# Autodesk Inventor assembly: assembled-antenna
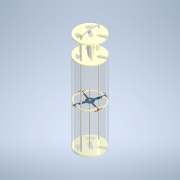
[picture p0: Inventor's stored thumbnail of the model, 180x180]
Saved by Autodesk Inventor 2021 (Build 250183000, 183)
## iProperties
Created: 2020-09-03
Part Number: assembled-antenna
Document SubType Name: Assembly
Designer: dsouthall
Author: dsouthall
## iProperties of the stored document inice_bottom.ipt
Created: 2020-11-16
Part Number: inice_bottom
Material: Generic
Document SubType Name: Modeling
Designer: dsouthall
Density: 1 g/cm^3
Appearance: Default
Author: dsouthall
Revision Number: ANY
## iProperties of the stored document inice_top.ipt
Created: 2020-11-16
Part Number: inice_top
Material: Generic
Document SubType Name: Modeling
Designer: dsouthall
Density: 1 g/cm^3
Appearance: Default
Author: dsouthall
Revision Number: ANY
## iProperties of the stored document front_end_box.iam
Created: 2020-11-16
Part Number: front_end_box
Description: STEP AP203
Document SubType Name: Assembly
Designer: dsouthall
Sending System: SolidWorks 2014
Preprocessor: SwSTEP 2.0
Title: front_end_box.STEP
Revision Number: ANY
## iProperties of the stored document fake_sma_with_cable.ipt
Created: 2020-11-16
Part Number: fake_sma_with_cable
Material: Generic
Document SubType Name: Modeling
Designer: dsouthall
Density: 1 g/cm^3
Appearance: Default
Author: dsouthall
Revision Number: ANY
## Documents named in this file (16)
- C:\Users\dsouthall\OneDrive - The University of Chicago\Hpol\hpol-prototype\design\Quad-Slot\Model 8 in\assembled-closed-antenna.iam
- C:\Users\dsouthall\OneDrive - The University of Chicago\Hpol\hpol-prototype\design\Quad-Slot\Model 8 in\assembled-feed.iam
- C:\Users\dsouthall\OneDrive - The University of Chicago\Hpol\hpol-prototype\design\Quad-Slot\Model 8 in\source\92141A003_TYPE 18-8 STAINLESS STEEL FLAT WASHER\92141A003_TYPE 18-8 STAINLESS STEEL FLAT WASHER.ipt
- C:\Users\dsouthall\OneDrive - The University of Chicago\Hpol\hpol-prototype\design\Quad-Slot\Model 8 in\source\96877A118_18-8 SS 82 DEG FLAT HEAD PHIL MACHINE SCREW\96877A118_18-8 SS 82 DEG FLAT HEAD PHIL MACHINE SCREW.ipt
- C:\Users\dsouthall\OneDrive - The University of Chicago\Hpol\hpol-prototype\design\Quad-Slot\Model 8 in\source\91841A003_TYPE 18-8 STAINLESS STEEL HEX NUT\91841A003_TYPE 18-8 STAINLESS STEEL HEX NUT.ipt
- C:\Users\dsouthall\OneDrive - The University of Chicago\Hpol\hpol-prototype\design\Quad-Slot\Model 8 in\source\my_faceplate.ipt
- C:\Users\dsouthall\OneDrive - The University of Chicago\Hpol\hpol-prototype\design\Quad-Slot\Model 8 in\source\my can\can_closed.ipt
- C:\Users\dsouthall\OneDrive - The University of Chicago\Hpol\hpol-prototype\design\Quad-Slot\Model 8 in\source\End Cap.ipt
- C:\Users\dsouthall\OneDrive - The University of Chicago\Hpol\hpol-prototype\design\Quad-Slot\Model 8 in\source\Short Support.ipt
- **C:\Users\dsouthall\OneDrive - The University of Chicago\Hpol\hpol-prototype\design\Quad-Slot\Model 8 in\assembled-closed-antenna.iam*LocalDocs*xAaaaamdaAaaaaaaaAaaaaxhxFa*front_end_box.iam
- C:\Users\dsouthall\OneDrive - The University of Chicago\Hpol\hpol-prototype\design\Quad-Slot\Model 8 in\source\rope.ipt
- C:\Users\dsouthall\OneDrive - The University of Chicago\Hpol\hpol-prototype\design\Quad-Slot\Model 8 in\source\99362A200_TAPPING INSERTS FOR PLASTICS\99362A200_TAPPING INSERTS FOR PLASTICS.ipt
- **C:\Users\dsouthall\OneDrive - The University of Chicago\Hpol\hpol-prototype\design\Quad-Slot\Model 8 in\assembled-closed-antenna.iam*LocalDocs*xAaaaamaaAaaaaaaaAaaaq5zb4b*inice_bottom.ipt
- **C:\Users\dsouthall\OneDrive - The University of Chicago\Hpol\hpol-prototype\design\Quad-Slot\Model 8 in\assembled-closed-antenna.iam*LocalDocs*xAaaaacaaAaaaaaaaAaaaqa3yKc*inice_top.ipt
- **C:\Users\dsouthall\OneDrive - The University of Chicago\Hpol\hpol-prototype\design\Quad-Slot\Model 8 in\assembled-closed-antenna.iam*LocalDocs*xAaaaq4aaAaaaaaaaAaaaqf0qEa*fake_sma_with_cable.ipt
- C:\Users\dsouthall\OneDrive - The University of Chicago\Hpol\hpol-prototype\design\Quad-Slot\Model 8 in\source\front_end_box.STEP
## Components (37 placed, 11 different names)
1. can_closed:1 — Insert:25, Insert:26, Insert:37, Insert:38, Mate:4, Mate:5, Flush:1, Angle:4, Angle:5, Insert:39, Insert:40, Angle:8
2. my_faceplate:1 — Insert:37, Angle:3
3. my_faceplate:2 — Insert:38, Angle:3
4. assembled-feed:1 [sub-assembly] — Mate:5, Flush:1, Angle:4, Angle:5
5. End Cap:1 — Angle:6, Insert:39, Insert:45, Insert:46
6. End Cap:2 — Angle:6, Insert:40, Insert:41, Insert:42, Insert:43, Angle:7, Mate:7, Angle:8
7. End Cap:3 — Insert:44, Mate:6, Angle:7, Mate:8, Tangent:1, Insert:47
8. Short Support:1 — Insert:41, Insert:44
9. Short Support:2 — Insert:42, Mate:6
10. Short Support:3 — Insert:43
11. front_end_box:1 [sub-assembly] — Mate:7, Mate:8, Tangent:1
12. rope:1 — Insert:45, Insert:46
13. 99362A200_TAPPING INSERTS FOR PLASTICS:1 — Insert:47
14. 92141A003_TYPE 18-8 STAINLESS STEEL FLAT WASHER:12 — Insert:35, Insert:36
15. 91841A003_TYPE 18-8 STAINLESS STEEL HEX NUT:3 — Insert:36
16. 96877A118_18-8 SS 82 DEG FLAT HEAD PHIL MACHINE SCREW:3 — Insert:26, Insert:35
17. 92141A003_TYPE 18-8 STAINLESS STEEL FLAT WASHER:13
18. 91841A003_TYPE 18-8 STAINLESS STEEL HEX NUT:7
19. 96877A118_18-8 SS 82 DEG FLAT HEAD PHIL MACHINE SCREW:7
20. 92141A003_TYPE 18-8 STAINLESS STEEL FLAT WASHER:14
21. 91841A003_TYPE 18-8 STAINLESS STEEL HEX NUT:8
22. 96877A118_18-8 SS 82 DEG FLAT HEAD PHIL MACHINE SCREW:8
23. 92141A003_TYPE 18-8 STAINLESS STEEL FLAT WASHER:15
24. 91841A003_TYPE 18-8 STAINLESS STEEL HEX NUT:9
25. 96877A118_18-8 SS 82 DEG FLAT HEAD PHIL MACHINE SCREW:9
26. 92141A003_TYPE 18-8 STAINLESS STEEL FLAT WASHER:11 — Insert:33, Insert:34
27. 91841A003_TYPE 18-8 STAINLESS STEEL HEX NUT:4 — Insert:34
28. 96877A118_18-8 SS 82 DEG FLAT HEAD PHIL MACHINE SCREW:4 — Insert:25, Insert:33
29. 92141A003_TYPE 18-8 STAINLESS STEEL FLAT WASHER:16
30. 91841A003_TYPE 18-8 STAINLESS STEEL HEX NUT:10
31. 96877A118_18-8 SS 82 DEG FLAT HEAD PHIL MACHINE SCREW:10
32. 92141A003_TYPE 18-8 STAINLESS STEEL FLAT WASHER:17
33. 91841A003_TYPE 18-8 STAINLESS STEEL HEX NUT:11
34. 96877A118_18-8 SS 82 DEG FLAT HEAD PHIL MACHINE SCREW:11
35. 92141A003_TYPE 18-8 STAINLESS STEEL FLAT WASHER:18
36. 91841A003_TYPE 18-8 STAINLESS STEEL HEX NUT:12
37. 96877A118_18-8 SS 82 DEG FLAT HEAD PHIL MACHINE SCREW:12
## Component patterns: (4 elements, first: 92141A003_TYPE 18-8 STAINLESS STEEL FLAT WASHER:12 + 91841A003_TYPE 18-8 STAINLESS STEEL HEX NUT:3 + 96877A118_18-8 SS 82 DEG FLAT HEAD PHIL MACHINE SCREW:3), (4 elements, first: 92141A003_TYPE 18-8 STAINLESS STEEL FLAT WASHER:11 + 91841A003_TYPE 18-8 STAINLESS STEEL HEX NUT:4 + 96877A118_18-8 SS 82 DEG FLAT HEAD PHIL MACHINE SCREW:4)
## Relationships (30: Insert 17, Angle 6, Mate 5, Flush 1, Tangent 1)
- Insert:25: can_closed:1 ↔ 96877A118_18-8 SS 82 DEG FLAT HEAD PHIL MACHINE SCREW:4
- Insert:26: can_closed:1 ↔ 96877A118_18-8 SS 82 DEG FLAT HEAD PHIL MACHINE SCREW:3
- Insert:33 (-2.54 mm): 92141A003_TYPE 18-8 STAINLESS STEEL FLAT WASHER:11 ↔ 96877A118_18-8 SS 82 DEG FLAT HEAD PHIL MACHINE SCREW:4
- Insert:34: 92141A003_TYPE 18-8 STAINLESS STEEL FLAT WASHER:11 ↔ 91841A003_TYPE 18-8 STAINLESS STEEL HEX NUT:4
- Insert:35 (-2.54 mm): 92141A003_TYPE 18-8 STAINLESS STEEL FLAT WASHER:12 ↔ 96877A118_18-8 SS 82 DEG FLAT HEAD PHIL MACHINE SCREW:3
- Insert:36: 92141A003_TYPE 18-8 STAINLESS STEEL FLAT WASHER:12 ↔ 91841A003_TYPE 18-8 STAINLESS STEEL HEX NUT:3
- Insert:37: can_closed:1 ↔ my_faceplate:1
- Insert:38 (-9.652 mm): can_closed:1 ↔ my_faceplate:2
- Angle:3 (0 deg): my_faceplate:1 ↔ my_faceplate:2
- Mate:4 (600 mm): can_closed:1
- Mate:5: can_closed:1 ↔ assembled-feed:1
- Flush:1 (-299.2 mm): can_closed:1 ↔ assembled-feed:1
- Angle:4 (0 deg): can_closed:1 ↔ assembled-feed:1
- Angle:5 (0 deg): can_closed:1 ↔ assembled-feed:1
- Angle:6 (0 deg): End Cap:1 ↔ End Cap:2
- Insert:39 (0.174 mm): can_closed:1 ↔ End Cap:1
- Insert:40 (-9.826 mm): can_closed:1 ↔ End Cap:2
- Insert:41: End Cap:2 ↔ Short Support:1
- Insert:42: End Cap:2 ↔ Short Support:2
- Insert:43: End Cap:2 ↔ Short Support:3
- Insert:44: End Cap:3 ↔ Short Support:1
- Mate:6: End Cap:3 ↔ Short Support:2
- Angle:7 (0 deg): End Cap:2 ↔ End Cap:3
- Mate:7 (6.35 mm): End Cap:2 ↔ front_end_box:1
- Mate:8 (1 mm): End Cap:3 ↔ front_end_box:1
- Angle:8 (0 deg): can_closed:1 ↔ End Cap:2
- Tangent:1: End Cap:3 ↔ front_end_box:1
- Insert:45: End Cap:1 ↔ rope:1
- Insert:46: End Cap:1 ↔ rope:1
- Insert:47 (1.651 mm): End Cap:3 ↔ 99362A200_TAPPING INSERTS FOR PLASTICS:1
